# Autodesk Inventor assembly: Microlab_Electrical_CAD
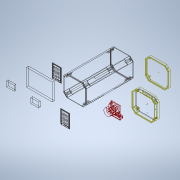
[picture p0: Inventor's stored thumbnail of the model, 180x180]
Saved by Autodesk Inventor 2022 (Build 260153000, 153)
## iProperties
Created: 2021-09-30
Part Number: Microlab_Electrical_CAD
Document SubType Name: Assembly
Designer: iss
Author: iss
## Documents named in this file (9)
- C:\Users\r8003\Downloads\Microlab_Electrical_CAD.iam
- C:\Users\r8003\Downloads\TPA6021A4EVM.ipt
- C:\Users\r8003\Downloads\AD9833Teyleten.ipt
- C:\Users\r8003\Downloads\MicroLab_Center_Shell.ipt
- C:\Users\r8003\Downloads\APS3008S-R.ipt
- C:\Users\r8003\Downloads\C329-SPI.ipt
- C:\Users\r8003\Downloads\MicroLab_Rear_Cover.ipt
- C:\Users\r8003\Downloads\MicroLab_Front_Cover.ipt
- C:\Users\r8003\Downloads\MicroLab_PCB_002.ipt
## Components (10 placed, 8 different names)
1. TPA6021A4EVM:1
2. AD9833Teyleten:1
3. MicroLab_Center_Shell:1
4. AD9833Teyleten:2
5. APS3008S-R:1
6. APS3008S-R:2
7. C329-SPI:1
8. MicroLab_Rear_Cover:1 — Mate:1, Mate:2, Mate:3
9. MicroLab_Front_Cover:1
10. MicroLab_PCB_002:1 — Mate:1, Mate:2, Mate:3
## Relationships (3: Mate 3)
- Mate:1: MicroLab_Rear_Cover:1 ↔ MicroLab_PCB_002:1
- Mate:2: MicroLab_Rear_Cover:1 ↔ MicroLab_PCB_002:1
- Mate:3: MicroLab_Rear_Cover:1 ↔ MicroLab_PCB_002:1
